# Autodesk Inventor assembly: demo
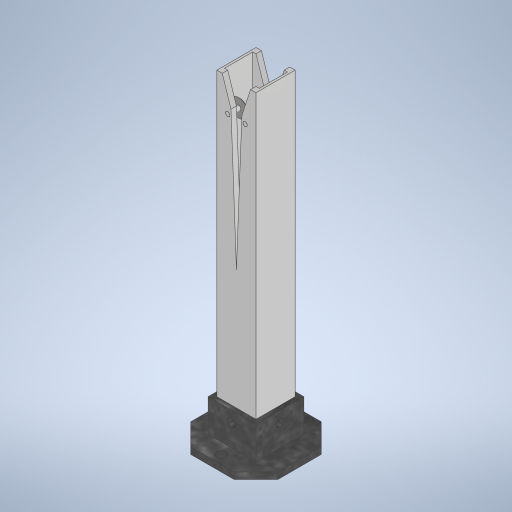
[picture p0: Inventor's stored thumbnail of the model, 512x512]
Saved by Autodesk Inventor 2024 (Build 280153000, 153)
## iProperties
Created: 2025-01-22
Part Number: demo
Document SubType Name: Assembly
Designer: 1412z
Author: 1412z
## Documents named in this file (5)
- C:\Users\1412z\OneDrive\デスクトップ\rdclab\harvesting_robot\harvesting_endeffector\demo_square_bar_endeffector\demo_square_bar_endeffector.iam
- C:\Users\1412z\OneDrive\デスクトップ\rdclab\harvesting_robot\harvesting_endeffector\demo_square_bar_endeffector\square_bar\square_bar.ipt
- C:\Users\1412z\OneDrive\デスクトップ\rdclab\harvesting_robot\harvesting_endeffector\demo_square_bar_endeffector\shaft\Φ2×18.ipt
- C:\Users\1412z\OneDrive\デスクトップ\rdclab\harvesting_robot\harvesting_endeffector\demo_square_bar_endeffector\blade\blade.ipt
- C:\Users\1412z\OneDrive\デスクトップ\rdclab\harvesting_robot\harvesting_endeffector\demo_square_bar_endeffector\square_bar_holder\square_ber_holder.ipt
## Components (6 placed, 4 different names)
1. square_bar:1 — 回転:1, 回転:2, 回転:3
2. blade:1 — リジッド:2
3. blade:2 — リジッド:1
4. Φ2×18:1 — 回転:1, リジッド:2
5. Φ2×18:2 — 回転:2, リジッド:1
6. square_ber_holder:1 — 回転:3
## Relationships (5: RevoluteJoint 3, WeldJoint 2)
- 回転:1 [RevoluteJoint]: square_bar:1 ↔ Φ2×18:1
- 回転:2 [RevoluteJoint]: square_bar:1 ↔ Φ2×18:2
- リジッド:1 [WeldJoint] (4 mm): blade:2 ↔ Φ2×18:2
- リジッド:2 [WeldJoint] (4.05 mm): blade:1 ↔ Φ2×18:1
- 回転:3 [RevoluteJoint]: square_bar:1 ↔ square_ber_holder:1
